# Autodesk Inventor assembly: FinalAssembly
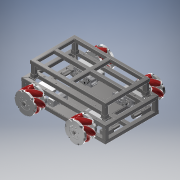
[picture p0: Inventor's stored thumbnail of the model, 180x180]
Saved by Autodesk Inventor 2018 (Build 220112000, 112)
## iProperties
Created: 2018-05-29
Part Number: FinalAssembly
Document SubType Name: Assembly
Designer: P136265
Author: P136265
## Documents named in this file (23)
- C:\Users\P136265\Documents\GitHub\mecanum-cad\FinalAssembly.iam
- C:\Users\P136265\Documents\GitHub\mecanum-cad\MecanumFrame2.iam
- C:\Users\P136265\Documents\GitHub\mecanum-cad\BearingHousing.iam
- C:\Users\P136265\Documents\GitHub\mecanum-cad\WheelShaft.ipt
- C:\Users\P136265\Documents\Inventor\Content Center Files\R2018\en-US\AS 1110\AS 1110 - M8 x 50.ipt
- C:\Users\P136265\Documents\Inventor\Content Center Files\R2018\en-US\AS 1112 (2)\AS 1112 - M8  Type 8.ipt
- C:\Users\P136265\Documents\GitHub\mecanum-cad\WheelKey.ipt
- C:\Users\P136265\Documents\GitHub\mecanum-cad\PulleyKey.ipt
- C:\Users\P136265\Documents\GitHub\mecanum-cad\Mecanum_Assembly.iam
- C:\Users\P136265\Documents\GitHub\mecanum-cad\LiftBase.ipt
- C:\Users\P136265\Documents\GitHub\mecanum-cad\mount.ipt
- C:\Users\P136265\Documents\GitHub\mecanum-cad\Nema 23 Stepper Motor Bipolar L=56mm w Gear Ratio 41 Planetary Gearbox.ipt
- C:\Users\P136265\Documents\GitHub\mecanum-cad\Synchronous Belt1.ipt
- C:\Users\P136265\Documents\GitHub\mecanum-cad\Synchronous Pulley21.ipt
- C:\Users\P136265\Documents\GitHub\mecanum-cad\Synchronous Pulley11.ipt
- C:\Users\P136265\Documents\Inventor\Content Center Files\R2018\en-US\BS EN 24035\ISO 4035 - M20BS EN.ipt
- C:\Users\P136265\Documents\Inventor\Content Center Files\R2018\en-US\BS EN 24035\ISO 4035 - M12BS EN.ipt
- C:\Users\P136265\Documents\GitHub\mecanum-cad\TS-58GZ868D_Open.ipt
- C:\Users\P136265\Documents\GitHub\mecanum-cad\12mm Ball Screw.ipt
- C:\Users\P136265\Documents\GitHub\mecanum-cad\16mm Lead Nut.ipt
- C:\Users\P136265\Documents\GitHub\mecanum-cad\LiftPlate.iam
- C:\Users\P136265\Documents\GitHub\mecanum-cad\LiftPlate_Mount.ipt
- C:\Users\P136265\Documents\Inventor\Content Center Files\R2018\en-US\AS 1110\AS 1110 - M3 x 6.ipt
## Components (119 placed, 22 different names)
1. MecanumFrame2:1 [sub-assembly] — Mate:1, Mate:2, Mate:3, Mate:4, Mate:5, Mate:6, Mate:7, Mate:8, Mate:9, Mate:10, Mate:11, Mate:12, Mate:13, Mate:14, Mate:15, Mate:24, Mate:25, Mate:26, Mate:27, Mate:28, Mate:29, Mate:30, Mate:31, Mate:32, Mate:33, Mate:34, Mate:35, Mate:36, Mate:37, Insert:1, Mate:38, Mate:39, Mate:40, Mate:41, Insert:2, Insert:3, Insert:4, Insert:5, Insert:6, Insert:7, Mate:106, Mate:107, Mate:108, Angle:5, Angle:8, Mate:185, Mate:186, Mate:187, Mate:188, Angle:15, Mate:191, Mate:192
2. BearingHousing:1 [sub-assembly] — Mate:4, Mate:5, Mate:6, Mate:16, Mate:17, Mate:43, Mate:45, Mate:47, Mate:49, Mate:156
3. BearingHousing:2 [sub-assembly] — Mate:7, Mate:8, Mate:9, Mate:18, Mate:19, Mate:51, Mate:53, Mate:55, Mate:57, Mate:154
4. BearingHousing:3 [sub-assembly] — Mate:10, Mate:11, Mate:12, Mate:20, Mate:21, Mate:67, Mate:69, Mate:71, Mate:73, Mate:150
5. BearingHousing:4 [sub-assembly] — Mate:13, Mate:14, Mate:15, Mate:22, Mate:23, Mate:59, Mate:61, Mate:63, Mate:65, Mate:152
6. WheelShaft:1 — Mate:16, Mate:17, Mate:77, Mate:78, Mate:79, Mate:89, Mate:90, Mate:91, Mate:98, Mate:99, Mate:134, Mate:137, Flush:8, Mate:141, Mate:155, Mate:157
7. WheelShaft:2 — Mate:18, Mate:19, Mate:74, Mate:75, Mate:76, Mate:92, Mate:93, Mate:94, Mate:100, Mate:101, Mate:131, Mate:136, Flush:7, Mate:143, Mate:153, Mate:163
8. WheelShaft:3 — Mate:20, Mate:21, Mate:83, Mate:84, Mate:85, Mate:86, Mate:87, Mate:88, Mate:104, Mate:105, Mate:116, Mate:118, Flush:1, Mate:147, Mate:149, Mate:159
9. WheelShaft:4 — Mate:22, Mate:23, Mate:80, Mate:81, Mate:82, Mate:95, Mate:96, Mate:97, Mate:102, Mate:103, Mate:129, Mate:135, Flush:6, Mate:145, Mate:151, Mate:161
10. AS 1110 - Metric M8 x 50:1 — Mate:24, Mate:25, Mate:42
11. AS 1110 - Metric M8 x 50:2 — Mate:26, Mate:27, Mate:44
12. AS 1110 - Metric M8 x 50:3 — Mate:28, Mate:29, Mate:50
13. AS 1110 - Metric M8 x 50:4 — Mate:30, Mate:31, Mate:54
14. AS 1110 - Metric M8 x 50:5 — Mate:32, Mate:33, Mate:56
15. AS 1110 - Metric M8 x 50:6 — Mate:34, Mate:35, Mate:52
16. AS 1110 - Metric M8 x 50:7 — Mate:36, Mate:37, Mate:46
17. AS 1110 - Metric M8 x 50:8 — Insert:1, Mate:48
18. AS 1110 - Metric M8 x 50:9 — Mate:38, Mate:39, Mate:72
19. AS 1110 - Metric M8 x 50:10 — Mate:40, Mate:41, Mate:68
20. AS 1110 - Metric M8 x 50:11 — Insert:2, Mate:64
21. AS 1110 - Metric M8 x 50:12 — Insert:3, Mate:60
22. AS 1110 - Metric M8 x 50:13 — Insert:4, Mate:58
23. AS 1110 - Metric M8 x 50:14 — Insert:5, Mate:62
24. AS 1110 - Metric M8 x 50:15 — Insert:6, Mate:66
25. AS 1110 - Metric M8 x 50:16 — Insert:7, Mate:70
26. AS 1112 (2) - Metric M8  Type 8:1 — Mate:42, Mate:43
27. AS 1112 (2) - Metric M8  Type 8:2 — Mate:44, Mate:45
28. AS 1112 (2) - Metric M8  Type 8:3 — Mate:46, Mate:47
29. AS 1112 (2) - Metric M8  Type 8:4 — Mate:48, Mate:49
30. AS 1112 (2) - Metric M8  Type 8:5 — Mate:50, Mate:51
31. AS 1112 (2) - Metric M8  Type 8:6 — Mate:52, Mate:53
32. AS 1112 (2) - Metric M8  Type 8:7 — Mate:54, Mate:55
33. AS 1112 (2) - Metric M8  Type 8:8 — Mate:56, Mate:57
34. AS 1112 (2) - Metric M8  Type 8:9 — Mate:58, Mate:59
35. AS 1112 (2) - Metric M8  Type 8:10 — Mate:60, Mate:61
36. AS 1112 (2) - Metric M8  Type 8:11 — Mate:62, Mate:63
37. AS 1112 (2) - Metric M8  Type 8:12 — Mate:64, Mate:65
38. AS 1112 (2) - Metric M8  Type 8:13 — Mate:66, Mate:67
39. AS 1112 (2) - Metric M8  Type 8:14 — Mate:68, Mate:69
40. AS 1112 (2) - Metric M8  Type 8:15 — Mate:70, Mate:71
41. AS 1112 (2) - Metric M8  Type 8:16 — Mate:72, Mate:73
42. WheelKey:1 — Mate:74, Mate:75, Mate:76, Angle:2
43. WheelKey:2 — Mate:77, Mate:78, Mate:79, Angle:1
44. WheelKey:3 — Mate:80, Mate:81, Mate:82, Angle:3
45. WheelKey:4 — Mate:83, Mate:84, Mate:85, Angle:4
46. PulleyKey:1 — Mate:86, Mate:87, Mate:88, Angle:6
47. PulleyKey:2 — Mate:89, Mate:90, Mate:91, Angle:9
48. PulleyKey:3 — Mate:92, Mate:93, Mate:94, Angle:10
49. PulleyKey:4 — Mate:95, Mate:96, Mate:97, Angle:11
50. Mecanum_Assembly:1 [sub-assembly] — Mate:98, Angle:1, Mate:99, Mate:142
51. Mecanum_Assembly:2 [sub-assembly] — Mate:100, Angle:2, Mate:101, Mate:144
52. Mecanum_Assembly:3 [sub-assembly] — Mate:104, Angle:4, Mate:105, Mate:148
53. Mecanum_Assembly:4 [sub-assembly] — Mate:102, Angle:3, Mate:103, Mate:146
54. LiftBase:1 — Mate:106, Mate:107, Mate:108, Mate:109, Mate:110, Mate:111, Mate:112, Mate:214, Mate:216, Mate:218, Mate:220, Mate:222, Mate:224, Mate:226, Mate:228, Mate:230, Mate:232, Mate:234, Mate:236, Mate:238, Mate:240, Mate:242, Mate:244
55. mount:1 — Mate:109, Mate:126, Mate:127, Mate:128, Mate:223, Mate:225, Mate:227, Mate:229
56. mount:2 — Mate:110, Mate:120, Mate:121, Mate:122, Mate:239, Mate:241, Mate:243, Mate:245
57. mount:3 — Mate:111, Mate:123, Mate:124, Mate:125, Mate:215, Mate:217, Mate:219, Mate:221
58. mount:4 — Mate:112, Mate:113, Mate:114, Mate:115, Mate:231, Mate:233, Mate:235, Mate:237
59. Nema 23 Stepper Motor Bipolar L=56mm w Gear Ratio 41 Planetary Gearbox:1 — Mate:113, Mate:114, Mate:115, Angle:5, Mate:117, Mate:119, Flush:3, Flush:4
60. Nema 23 Stepper Motor Bipolar L=56mm w Gear Ratio 41 Planetary Gearbox:2 — Mate:123, Mate:124, Mate:125, Flush:5, Mate:133, Mate:140, Flush:16
61. Nema 23 Stepper Motor Bipolar L=56mm w Gear Ratio 41 Planetary Gearbox:3 — Mate:126, Mate:127, Mate:128, Angle:8, Mate:132, Flush:5, Mate:139
62. Nema 23 Stepper Motor Bipolar L=56mm w Gear Ratio 41 Planetary Gearbox:4 — Mate:120, Mate:121, Mate:122, Flush:4, Mate:130, Mate:138
63. Synchronous Belt:1 — Mate:116, Mate:117, Flush:14
64. Synchronous Belt:2 — Mate:131, Mate:132, Flush:12
65. Synchronous Belt:3 — Mate:133, Mate:134, Flush:15
66. Synchronous Belt:4 — Mate:129, Mate:130, Flush:13
67. Synchronous Pulley2:1 — Mate:118, Angle:6, Flush:1, Angle:7, Flush:2, Flush:14, Mate:160
68. Synchronous Pulley2:2 — Mate:135, Flush:6, Angle:11, Flush:9, Angle:13, Mate:162
69. Synchronous Pulley2:3 — Mate:136, Flush:7, Angle:10, Flush:10, Angle:14, Mate:164
70. Synchronous Pulley2:4 — Mate:137, Flush:8, Angle:9, Flush:11, Angle:12, Flush:15, Mate:158
71. Synchronous Pulley1:1 — Mate:119, Angle:7, Flush:2, Flush:3
72. Synchronous Pulley1:2 — Mate:139, Flush:10, Angle:14, Flush:12
73. Synchronous Pulley1:3 — Mate:140, Flush:11, Angle:12, Flush:16
74. Synchronous Pulley1:4 — Mate:138, Flush:9, Angle:13, Flush:13
75. BS EN 24035 - Metric M20:1 — Mate:141, Mate:142
76. BS EN 24035 - Metric M20:2 — Mate:143, Mate:144
77. BS EN 24035 - Metric M20:3 — Mate:145, Mate:146
78. BS EN 24035 - Metric M20:4 — Mate:147, Mate:148
79. BS EN 24035 - Metric M20:5 — Mate:149, Mate:150
80. BS EN 24035 - Metric M20:6 — Mate:151, Mate:152
81. BS EN 24035 - Metric M20:7 — Mate:153, Mate:154
82. BS EN 24035 - Metric M20:8 — Mate:155, Mate:156
83. BS EN 24035 - Metric M12:1 — Mate:157, Mate:158
84. BS EN 24035 - Metric M12:2 — Mate:159, Mate:160
85. BS EN 24035 - Metric M12:3 — Mate:161, Mate:162
86. BS EN 24035 - Metric M12:4 — Mate:163, Mate:164
87. TS-58GZ868D_Open:1 — Mate:165, Flush:19
88. TS-58GZ868D_Open:2 — Mate:166, Mate:169
89. TS-58GZ868D_Open:3 — Mate:167, Flush:18
90. TS-58GZ868D_Open:4 — Mate:168, Flush:17
91. 12mm Ball Screw:1 — Mate:165, Flush:19, Mate:170, Flush:20, Mate:185
92. 12mm Ball Screw:2 — Mate:166, Mate:169, Mate:171, Flush:23, Mate:186
93. 12mm Ball Screw:3 — Mate:167, Flush:18, Mate:172, Flush:21, Mate:187
94. 12mm Ball Screw:4 — Mate:168, Flush:17, Mate:173, Flush:22, Mate:188
95. 16mm Lead Nut:1 — Mate:170, Flush:20, Flush:26, Flush:27, Mate:207, Mate:208
96. 16mm Lead Nut:2 — Mate:171, Flush:23, Flush:25, Flush:27, Mate:196, Mate:197
97. 16mm Lead Nut:3 — Mate:172, Flush:21, Flush:24, Flush:26, Mate:209, Mate:210
98. 16mm Lead Nut:4 — Mate:173, Flush:22, Flush:24, Flush:25, Mate:211, Mate:212, Mate:213
99. LiftPlate:1 [sub-assembly] — Angle:15, Mate:191, Mate:192, Mate:193, Mate:194, Mate:195, Mate:198, Mate:199, Mate:200, Mate:201, Mate:202, Mate:203, Mate:204, Mate:205, Mate:206
100. LiftPlate_Mount:1 — Mate:193, Mate:194, Mate:195, Mate:196, Mate:197
101. LiftPlate_Mount:2 — Mate:201, Mate:202, Mate:203, Mate:209, Mate:210
102. LiftPlate_Mount:3 — Mate:204, Mate:205, Mate:206, Mate:207, Mate:208
103. LiftPlate_Mount:4 — Mate:198, Mate:199, Mate:200, Mate:211, Mate:212, Mate:213
104. AS 1110 - Metric M3 x 6:1 — Mate:214, Mate:215
105. AS 1110 - Metric M3 x 6:2 — Mate:216, Mate:217
106. AS 1110 - Metric M3 x 6:3 — Mate:218, Mate:219
107. AS 1110 - Metric M3 x 6:4 — Mate:220, Mate:221
108. AS 1110 - Metric M3 x 6:5 — Mate:222, Mate:223
109. AS 1110 - Metric M3 x 6:6 — Mate:224, Mate:225
110. AS 1110 - Metric M3 x 6:7 — Mate:226, Mate:227
111. AS 1110 - Metric M3 x 6:8 — Mate:228, Mate:229
112. AS 1110 - Metric M3 x 6:9 — Mate:230, Mate:231
113. AS 1110 - Metric M3 x 6:10 — Mate:232, Mate:233
114. AS 1110 - Metric M3 x 6:11 — Mate:234, Mate:235
115. AS 1110 - Metric M3 x 6:12 — Mate:236, Mate:237
116. AS 1110 - Metric M3 x 6:13 — Mate:238, Mate:239
117. AS 1110 - Metric M3 x 6:14 — Mate:240, Mate:241
118. AS 1110 - Metric M3 x 6:15 — Mate:242, Mate:243
119. AS 1110 - Metric M3 x 6:16 — Mate:244, Mate:245
## Relationships (281: Mate 232, Flush 27, Angle 15, Insert 7)
- Mate:1: MecanumFrame2:1
- Mate:2: MecanumFrame2:1
- Mate:3: MecanumFrame2:1
- Mate:4: MecanumFrame2:1 ↔ BearingHousing:1
- Mate:5: MecanumFrame2:1 ↔ BearingHousing:1
- Mate:6: MecanumFrame2:1 ↔ BearingHousing:1
- Mate:7: MecanumFrame2:1 ↔ BearingHousing:2
- Mate:8: MecanumFrame2:1 ↔ BearingHousing:2
- Mate:9: MecanumFrame2:1 ↔ BearingHousing:2
- Mate:10: MecanumFrame2:1 ↔ BearingHousing:3
- Mate:11: MecanumFrame2:1 ↔ BearingHousing:3
- Mate:12: MecanumFrame2:1 ↔ BearingHousing:3
- Mate:13: MecanumFrame2:1 ↔ BearingHousing:4
- Mate:14: MecanumFrame2:1 ↔ BearingHousing:4
- Mate:15: MecanumFrame2:1 ↔ BearingHousing:4
- Mate:16: BearingHousing:1 ↔ WheelShaft:1
- Mate:17: BearingHousing:1 ↔ WheelShaft:1
- Mate:18: BearingHousing:2 ↔ WheelShaft:2
- Mate:19: BearingHousing:2 ↔ WheelShaft:2
- Mate:20: BearingHousing:3 ↔ WheelShaft:3
- Mate:21: BearingHousing:3 ↔ WheelShaft:3
- Mate:22: BearingHousing:4 ↔ WheelShaft:4
- Mate:23: BearingHousing:4 ↔ WheelShaft:4
- Mate:24: MecanumFrame2:1 ↔ AS 1110 - Metric M8 x 50:1
- Mate:25: MecanumFrame2:1 ↔ AS 1110 - Metric M8 x 50:1
- Mate:26: MecanumFrame2:1 ↔ AS 1110 - Metric M8 x 50:2
- Mate:27: MecanumFrame2:1 ↔ AS 1110 - Metric M8 x 50:2
- Mate:28: MecanumFrame2:1 ↔ AS 1110 - Metric M8 x 50:3
- Mate:29: MecanumFrame2:1 ↔ AS 1110 - Metric M8 x 50:3
- Mate:30: MecanumFrame2:1 ↔ AS 1110 - Metric M8 x 50:4
- Mate:31: MecanumFrame2:1 ↔ AS 1110 - Metric M8 x 50:4
- Mate:32: MecanumFrame2:1 ↔ AS 1110 - Metric M8 x 50:5
- Mate:33: MecanumFrame2:1 ↔ AS 1110 - Metric M8 x 50:5
- Mate:34: MecanumFrame2:1 ↔ AS 1110 - Metric M8 x 50:6
- Mate:35: MecanumFrame2:1 ↔ AS 1110 - Metric M8 x 50:6
- Mate:36: MecanumFrame2:1 ↔ AS 1110 - Metric M8 x 50:7
- Mate:37: MecanumFrame2:1 ↔ AS 1110 - Metric M8 x 50:7
- Insert:1: MecanumFrame2:1 ↔ AS 1110 - Metric M8 x 50:8
- Mate:38: MecanumFrame2:1 ↔ AS 1110 - Metric M8 x 50:9
- Mate:39: MecanumFrame2:1 ↔ AS 1110 - Metric M8 x 50:9
- Mate:40: MecanumFrame2:1 ↔ AS 1110 - Metric M8 x 50:10
- Mate:41: MecanumFrame2:1 ↔ AS 1110 - Metric M8 x 50:10
- Insert:2: MecanumFrame2:1 ↔ AS 1110 - Metric M8 x 50:11
- Insert:3: MecanumFrame2:1 ↔ AS 1110 - Metric M8 x 50:12
- Insert:4: MecanumFrame2:1 ↔ AS 1110 - Metric M8 x 50:13
- Insert:5: MecanumFrame2:1 ↔ AS 1110 - Metric M8 x 50:14
- Insert:6: MecanumFrame2:1 ↔ AS 1110 - Metric M8 x 50:15
- Insert:7: MecanumFrame2:1 ↔ AS 1110 - Metric M8 x 50:16
- Mate:42: AS 1110 - Metric M8 x 50:1 ↔ AS 1112 (2) - Metric M8  Type 8:1
- Mate:43: BearingHousing:1 ↔ AS 1112 (2) - Metric M8  Type 8:1
- Mate:44: AS 1110 - Metric M8 x 50:2 ↔ AS 1112 (2) - Metric M8  Type 8:2
- Mate:45: BearingHousing:1 ↔ AS 1112 (2) - Metric M8  Type 8:2
- Mate:46: AS 1110 - Metric M8 x 50:7 ↔ AS 1112 (2) - Metric M8  Type 8:3
- Mate:47: BearingHousing:1 ↔ AS 1112 (2) - Metric M8  Type 8:3
- Mate:48: AS 1110 - Metric M8 x 50:8 ↔ AS 1112 (2) - Metric M8  Type 8:4
- Mate:49: BearingHousing:1 ↔ AS 1112 (2) - Metric M8  Type 8:4
- Mate:50: AS 1110 - Metric M8 x 50:3 ↔ AS 1112 (2) - Metric M8  Type 8:5
- Mate:51: BearingHousing:2 ↔ AS 1112 (2) - Metric M8  Type 8:5
- Mate:52: AS 1110 - Metric M8 x 50:6 ↔ AS 1112 (2) - Metric M8  Type 8:6
- Mate:53: BearingHousing:2 ↔ AS 1112 (2) - Metric M8  Type 8:6
- Mate:54: AS 1110 - Metric M8 x 50:4 ↔ AS 1112 (2) - Metric M8  Type 8:7
- Mate:55: BearingHousing:2 ↔ AS 1112 (2) - Metric M8  Type 8:7
- Mate:56: AS 1110 - Metric M8 x 50:5 ↔ AS 1112 (2) - Metric M8  Type 8:8
- Mate:57: BearingHousing:2 ↔ AS 1112 (2) - Metric M8  Type 8:8
- Mate:58: AS 1110 - Metric M8 x 50:13 ↔ AS 1112 (2) - Metric M8  Type 8:9
- Mate:59: BearingHousing:4 ↔ AS 1112 (2) - Metric M8  Type 8:9
- Mate:60: AS 1110 - Metric M8 x 50:12 ↔ AS 1112 (2) - Metric M8  Type 8:10
- Mate:61: BearingHousing:4 ↔ AS 1112 (2) - Metric M8  Type 8:10
- Mate:62: AS 1110 - Metric M8 x 50:14 ↔ AS 1112 (2) - Metric M8  Type 8:11
- Mate:63: BearingHousing:4 ↔ AS 1112 (2) - Metric M8  Type 8:11
- Mate:64: AS 1110 - Metric M8 x 50:11 ↔ AS 1112 (2) - Metric M8  Type 8:12
- Mate:65: BearingHousing:4 ↔ AS 1112 (2) - Metric M8  Type 8:12
- Mate:66: AS 1110 - Metric M8 x 50:15 ↔ AS 1112 (2) - Metric M8  Type 8:13
- Mate:67: BearingHousing:3 ↔ AS 1112 (2) - Metric M8  Type 8:13
- Mate:68: AS 1110 - Metric M8 x 50:10 ↔ AS 1112 (2) - Metric M8  Type 8:14
- Mate:69: BearingHousing:3 ↔ AS 1112 (2) - Metric M8  Type 8:14
- Mate:70: AS 1110 - Metric M8 x 50:16 ↔ AS 1112 (2) - Metric M8  Type 8:15
- Mate:71: BearingHousing:3 ↔ AS 1112 (2) - Metric M8  Type 8:15
- Mate:72: AS 1110 - Metric M8 x 50:9 ↔ AS 1112 (2) - Metric M8  Type 8:16
- Mate:73: BearingHousing:3 ↔ AS 1112 (2) - Metric M8  Type 8:16
- Mate:74: WheelShaft:2 ↔ WheelKey:1
- Mate:75: WheelShaft:2 ↔ WheelKey:1
- Mate:76: WheelShaft:2 ↔ WheelKey:1
- Mate:77: WheelShaft:1 ↔ WheelKey:2
- Mate:78: WheelShaft:1 ↔ WheelKey:2
- Mate:79: WheelShaft:1 ↔ WheelKey:2
- Mate:80: WheelShaft:4 ↔ WheelKey:3
- Mate:81: WheelShaft:4 ↔ WheelKey:3
- Mate:82: WheelShaft:4 ↔ WheelKey:3
- Mate:83: WheelShaft:3 ↔ WheelKey:4
- Mate:84: WheelShaft:3 ↔ WheelKey:4
- Mate:85: WheelShaft:3 ↔ WheelKey:4
- Mate:86: WheelShaft:3 ↔ PulleyKey:1
- Mate:87: WheelShaft:3 ↔ PulleyKey:1
- Mate:88: WheelShaft:3 ↔ PulleyKey:1
- Mate:89: WheelShaft:1 ↔ PulleyKey:2
- Mate:90: WheelShaft:1 ↔ PulleyKey:2
- Mate:91: WheelShaft:1 ↔ PulleyKey:2
- Mate:92: WheelShaft:2 ↔ PulleyKey:3
- Mate:93: WheelShaft:2 ↔ PulleyKey:3
- Mate:94: WheelShaft:2 ↔ PulleyKey:3
- Mate:95: WheelShaft:4 ↔ PulleyKey:4
- Mate:96: WheelShaft:4 ↔ PulleyKey:4
- Mate:97: WheelShaft:4 ↔ PulleyKey:4
- Mate:98: WheelShaft:1 ↔ Mecanum_Assembly:1
- Angle:1 (0 deg): WheelKey:2 ↔ Mecanum_Assembly:1
- Mate:99: WheelShaft:1 ↔ Mecanum_Assembly:1
- Mate:100: WheelShaft:2 ↔ Mecanum_Assembly:2
- Angle:2 (0 deg): WheelKey:1 ↔ Mecanum_Assembly:2
- Mate:101: WheelShaft:2 ↔ Mecanum_Assembly:2
- Mate:102: WheelShaft:4 ↔ Mecanum_Assembly:4
- Angle:3 (0 deg): WheelKey:3 ↔ Mecanum_Assembly:4
- Mate:103: WheelShaft:4 ↔ Mecanum_Assembly:4
- Mate:104: WheelShaft:3 ↔ Mecanum_Assembly:3
- Angle:4 (0 deg): WheelKey:4 ↔ Mecanum_Assembly:3
- Mate:105: WheelShaft:3 ↔ Mecanum_Assembly:3
- Mate:106: MecanumFrame2:1 ↔ LiftBase:1
- Mate:107: MecanumFrame2:1 ↔ LiftBase:1
- Mate:108: MecanumFrame2:1 ↔ LiftBase:1
- Mate:109: LiftBase:1 ↔ mount:1
- Mate:110: LiftBase:1 ↔ mount:2
- Mate:111: LiftBase:1 ↔ mount:3
- Mate:112: LiftBase:1 ↔ mount:4
- Mate:113: mount:4 ↔ Nema 23 Stepper Motor Bipolar L=56mm w Gear Ratio 41 Planetary Gearbox:1
- Mate:114: mount:4 ↔ Nema 23 Stepper Motor Bipolar L=56mm w Gear Ratio 41 Planetary Gearbox:1
- Mate:115: mount:4 ↔ Nema 23 Stepper Motor Bipolar L=56mm w Gear Ratio 41 Planetary Gearbox:1
- Angle:5 (0 deg): MecanumFrame2:1 ↔ Nema 23 Stepper Motor Bipolar L=56mm w Gear Ratio 41 Planetary Gearbox:1
- Mate:116: WheelShaft:3 ↔ Synchronous Belt:1
- Mate:117: Nema 23 Stepper Motor Bipolar L=56mm w Gear Ratio 41 Planetary Gearbox:1 ↔ Synchronous Belt:1
- Mate:118: WheelShaft:3 ↔ Synchronous Pulley2:1
- Angle:6 (0 deg): PulleyKey:1 ↔ Synchronous Pulley2:1
- Flush:1 (10 mm): WheelShaft:3 ↔ Synchronous Pulley2:1
- Mate:119: Nema 23 Stepper Motor Bipolar L=56mm w Gear Ratio 41 Planetary Gearbox:1 ↔ Synchronous Pulley1:1
- Angle:7 (0 deg): Synchronous Pulley2:1 ↔ Synchronous Pulley1:1
- Flush:2: Synchronous Pulley2:1 ↔ Synchronous Pulley1:1
- Flush:3: Nema 23 Stepper Motor Bipolar L=56mm w Gear Ratio 41 Planetary Gearbox:1 ↔ Synchronous Pulley1:1
- Mate:120: mount:2 ↔ Nema 23 Stepper Motor Bipolar L=56mm w Gear Ratio 41 Planetary Gearbox:4
- Mate:121: mount:2 ↔ Nema 23 Stepper Motor Bipolar L=56mm w Gear Ratio 41 Planetary Gearbox:4
- Mate:122: mount:2 ↔ Nema 23 Stepper Motor Bipolar L=56mm w Gear Ratio 41 Planetary Gearbox:4
- Mate:123: mount:3 ↔ Nema 23 Stepper Motor Bipolar L=56mm w Gear Ratio 41 Planetary Gearbox:2
- Mate:124: mount:3 ↔ Nema 23 Stepper Motor Bipolar L=56mm w Gear Ratio 41 Planetary Gearbox:2
- Mate:125: mount:3 ↔ Nema 23 Stepper Motor Bipolar L=56mm w Gear Ratio 41 Planetary Gearbox:2
- Mate:126: mount:1 ↔ Nema 23 Stepper Motor Bipolar L=56mm w Gear Ratio 41 Planetary Gearbox:3
- Mate:127: mount:1 ↔ Nema 23 Stepper Motor Bipolar L=56mm w Gear Ratio 41 Planetary Gearbox:3
- Mate:128: mount:1 ↔ Nema 23 Stepper Motor Bipolar L=56mm w Gear Ratio 41 Planetary Gearbox:3
- Flush:4: Nema 23 Stepper Motor Bipolar L=56mm w Gear Ratio 41 Planetary Gearbox:1 ↔ Nema 23 Stepper Motor Bipolar L=56mm w Gear Ratio 41 Planetary Gearbox:4
- Mate:129: WheelShaft:4 ↔ Synchronous Belt:4
- Mate:130: Nema 23 Stepper Motor Bipolar L=56mm w Gear Ratio 41 Planetary Gearbox:4 ↔ Synchronous Belt:4
- Angle:8 (0 deg): MecanumFrame2:1 ↔ Nema 23 Stepper Motor Bipolar L=56mm w Gear Ratio 41 Planetary Gearbox:3
- Mate:131: WheelShaft:2 ↔ Synchronous Belt:2
- Mate:132: Nema 23 Stepper Motor Bipolar L=56mm w Gear Ratio 41 Planetary Gearbox:3 ↔ Synchronous Belt:2
- Flush:5: Nema 23 Stepper Motor Bipolar L=56mm w Gear Ratio 41 Planetary Gearbox:2 ↔ Nema 23 Stepper Motor Bipolar L=56mm w Gear Ratio 41 Planetary Gearbox:3
- Mate:133: Nema 23 Stepper Motor Bipolar L=56mm w Gear Ratio 41 Planetary Gearbox:2 ↔ Synchronous Belt:3
- Mate:134: WheelShaft:1 ↔ Synchronous Belt:3
- Mate:135: WheelShaft:4 ↔ Synchronous Pulley2:2
- Flush:6 (10 mm): WheelShaft:4 ↔ Synchronous Pulley2:2
- Mate:136: WheelShaft:2 ↔ Synchronous Pulley2:3
- Flush:7 (10 mm): WheelShaft:2 ↔ Synchronous Pulley2:3
- Mate:137: WheelShaft:1 ↔ Synchronous Pulley2:4
- Flush:8 (10 mm): WheelShaft:1 ↔ Synchronous Pulley2:4
- Angle:9 (0 deg): PulleyKey:2 ↔ Synchronous Pulley2:4
- Angle:10 (0 deg): PulleyKey:3 ↔ Synchronous Pulley2:3
- Angle:11 (0 deg): PulleyKey:4 ↔ Synchronous Pulley2:2
- Mate:138: Nema 23 Stepper Motor Bipolar L=56mm w Gear Ratio 41 Planetary Gearbox:4 ↔ Synchronous Pulley1:4
- Flush:9: Synchronous Pulley2:2 ↔ Synchronous Pulley1:4
- Mate:139: Nema 23 Stepper Motor Bipolar L=56mm w Gear Ratio 41 Planetary Gearbox:3 ↔ Synchronous Pulley1:2
- Flush:10: Synchronous Pulley2:3 ↔ Synchronous Pulley1:2
- Mate:140: Nema 23 Stepper Motor Bipolar L=56mm w Gear Ratio 41 Planetary Gearbox:2 ↔ Synchronous Pulley1:3
- Flush:11: Synchronous Pulley2:4 ↔ Synchronous Pulley1:3
- Angle:12 (0 deg): Synchronous Pulley2:4 ↔ Synchronous Pulley1:3
- Angle:13 (0 deg): Synchronous Pulley2:2 ↔ Synchronous Pulley1:4
- Angle:14 (0 deg): Synchronous Pulley2:3 ↔ Synchronous Pulley1:2
- Flush:12 (1.5 mm): Synchronous Belt:2 ↔ Synchronous Pulley1:2
- Flush:13 (1.5 mm): Synchronous Belt:4 ↔ Synchronous Pulley1:4
- Flush:14 (1.5 mm): Synchronous Belt:1 ↔ Synchronous Pulley2:1
- Flush:15 (1.5 mm): Synchronous Belt:3 ↔ Synchronous Pulley2:4
- Flush:16: Nema 23 Stepper Motor Bipolar L=56mm w Gear Ratio 41 Planetary Gearbox:2 ↔ Synchronous Pulley1:3
- Mate:141: WheelShaft:1 ↔ BS EN 24035 - Metric M20:1
- Mate:142: Mecanum_Assembly:1 ↔ BS EN 24035 - Metric M20:1
- Mate:143: WheelShaft:2 ↔ BS EN 24035 - Metric M20:2
- Mate:144: Mecanum_Assembly:2 ↔ BS EN 24035 - Metric M20:2
- Mate:145: WheelShaft:4 ↔ BS EN 24035 - Metric M20:3
- Mate:146: Mecanum_Assembly:4 ↔ BS EN 24035 - Metric M20:3
- Mate:147: WheelShaft:3 ↔ BS EN 24035 - Metric M20:4
- Mate:148: Mecanum_Assembly:3 ↔ BS EN 24035 - Metric M20:4
- Mate:149: WheelShaft:3 ↔ BS EN 24035 - Metric M20:5
- Mate:150: BearingHousing:3 ↔ BS EN 24035 - Metric M20:5
- Mate:151: WheelShaft:4 ↔ BS EN 24035 - Metric M20:6
- Mate:152: BearingHousing:4 ↔ BS EN 24035 - Metric M20:6
- Mate:153: WheelShaft:2 ↔ BS EN 24035 - Metric M20:7
- Mate:154: BearingHousing:2 ↔ BS EN 24035 - Metric M20:7
- Mate:155: WheelShaft:1 ↔ BS EN 24035 - Metric M20:8
- Mate:156: BearingHousing:1 ↔ BS EN 24035 - Metric M20:8
- Mate:157: WheelShaft:1 ↔ BS EN 24035 - Metric M12:1
- Mate:158: Synchronous Pulley2:4 ↔ BS EN 24035 - Metric M12:1
- Mate:159: WheelShaft:3 ↔ BS EN 24035 - Metric M12:2
- Mate:160: Synchronous Pulley2:1 ↔ BS EN 24035 - Metric M12:2
- Mate:161: WheelShaft:4 ↔ BS EN 24035 - Metric M12:3
- Mate:162: Synchronous Pulley2:2 ↔ BS EN 24035 - Metric M12:3
- Mate:163: WheelShaft:2 ↔ BS EN 24035 - Metric M12:4
- Mate:164: Synchronous Pulley2:3 ↔ BS EN 24035 - Metric M12:4
- Mate:165: TS-58GZ868D_Open:1 ↔ 12mm Ball Screw:1
- Mate:166: TS-58GZ868D_Open:2 ↔ 12mm Ball Screw:2
- Mate:167: TS-58GZ868D_Open:3 ↔ 12mm Ball Screw:3
- Mate:168: TS-58GZ868D_Open:4 ↔ 12mm Ball Screw:4
- Flush:17 (130 mm): TS-58GZ868D_Open:4 ↔ 12mm Ball Screw:4
- Flush:18 (130 mm): TS-58GZ868D_Open:3 ↔ 12mm Ball Screw:3
- Mate:169 (130 mm): TS-58GZ868D_Open:2 ↔ 12mm Ball Screw:2
- Flush:19 (130 mm): TS-58GZ868D_Open:1 ↔ 12mm Ball Screw:1
- Mate:170: 12mm Ball Screw:1 ↔ 16mm Lead Nut:1
- Mate:171: 12mm Ball Screw:2 ↔ 16mm Lead Nut:2
- Mate:172: 12mm Ball Screw:3 ↔ 16mm Lead Nut:3
- Mate:173: 12mm Ball Screw:4 ↔ 16mm Lead Nut:4
- Flush:20: 12mm Ball Screw:1 ↔ 16mm Lead Nut:1
- Flush:21: 12mm Ball Screw:3 ↔ 16mm Lead Nut:3
- Flush:22: 12mm Ball Screw:4 ↔ 16mm Lead Nut:4
- Flush:23: 12mm Ball Screw:2 ↔ 16mm Lead Nut:2
- Flush:24: 16mm Lead Nut:3 ↔ 16mm Lead Nut:4
- Flush:25: 16mm Lead Nut:2 ↔ 16mm Lead Nut:4
- Flush:26: 16mm Lead Nut:1 ↔ 16mm Lead Nut:3
- Flush:27: 16mm Lead Nut:1 ↔ 16mm Lead Nut:2
- Mate:185: MecanumFrame2:1 ↔ 12mm Ball Screw:1
- Mate:186: MecanumFrame2:1 ↔ 12mm Ball Screw:2
- Mate:187: MecanumFrame2:1 ↔ 12mm Ball Screw:3
- Mate:188: MecanumFrame2:1 ↔ 12mm Ball Screw:4
- Angle:15 (0 deg): MecanumFrame2:1 ↔ LiftPlate:1
- Mate:191 (7.5 mm): MecanumFrame2:1 ↔ LiftPlate:1
- Mate:192 (7.5 mm): MecanumFrame2:1 ↔ LiftPlate:1
- Mate:193: LiftPlate:1 ↔ LiftPlate_Mount:1
- Mate:194: LiftPlate:1 ↔ LiftPlate_Mount:1
- Mate:195: LiftPlate:1 ↔ LiftPlate_Mount:1
- Mate:196: 16mm Lead Nut:2 ↔ LiftPlate_Mount:1
- Mate:197: 16mm Lead Nut:2 ↔ LiftPlate_Mount:1
- Mate:198: LiftPlate:1 ↔ LiftPlate_Mount:4
- Mate:199: LiftPlate:1 ↔ LiftPlate_Mount:4
- Mate:200: LiftPlate:1 ↔ LiftPlate_Mount:4
- Mate:201: LiftPlate:1 ↔ LiftPlate_Mount:2
- Mate:202: LiftPlate:1 ↔ LiftPlate_Mount:2
- Mate:203: LiftPlate:1 ↔ LiftPlate_Mount:2
- Mate:204: LiftPlate:1 ↔ LiftPlate_Mount:3
- Mate:205: LiftPlate:1 ↔ LiftPlate_Mount:3
- Mate:206: LiftPlate:1 ↔ LiftPlate_Mount:3
- Mate:207: 16mm Lead Nut:1 ↔ LiftPlate_Mount:3
- Mate:208: 16mm Lead Nut:1 ↔ LiftPlate_Mount:3
- Mate:209: 16mm Lead Nut:3 ↔ LiftPlate_Mount:2
- Mate:210: 16mm Lead Nut:3 ↔ LiftPlate_Mount:2
- Mate:211: 16mm Lead Nut:4 ↔ LiftPlate_Mount:4
- Mate:212: 16mm Lead Nut:4 ↔ LiftPlate_Mount:4
- Mate:213: 16mm Lead Nut:4 ↔ LiftPlate_Mount:4
- Mate:214: LiftBase:1 ↔ AS 1110 - Metric M3 x 6:1
- Mate:215: mount:3 ↔ AS 1110 - Metric M3 x 6:1
- Mate:216: LiftBase:1 ↔ AS 1110 - Metric M3 x 6:2
- Mate:217: mount:3 ↔ AS 1110 - Metric M3 x 6:2
- Mate:218: LiftBase:1 ↔ AS 1110 - Metric M3 x 6:3
- Mate:219: mount:3 ↔ AS 1110 - Metric M3 x 6:3
- Mate:220: LiftBase:1 ↔ AS 1110 - Metric M3 x 6:4
- Mate:221: mount:3 ↔ AS 1110 - Metric M3 x 6:4
- Mate:222: LiftBase:1 ↔ AS 1110 - Metric M3 x 6:5
- Mate:223: mount:1 ↔ AS 1110 - Metric M3 x 6:5
- Mate:224: LiftBase:1 ↔ AS 1110 - Metric M3 x 6:6
- Mate:225: mount:1 ↔ AS 1110 - Metric M3 x 6:6
- Mate:226: LiftBase:1 ↔ AS 1110 - Metric M3 x 6:7
- Mate:227: mount:1 ↔ AS 1110 - Metric M3 x 6:7
- Mate:228: LiftBase:1 ↔ AS 1110 - Metric M3 x 6:8
- Mate:229: mount:1 ↔ AS 1110 - Metric M3 x 6:8
- Mate:230: LiftBase:1 ↔ AS 1110 - Metric M3 x 6:9
- Mate:231: mount:4 ↔ AS 1110 - Metric M3 x 6:9
- Mate:232: LiftBase:1 ↔ AS 1110 - Metric M3 x 6:10
- Mate:233: mount:4 ↔ AS 1110 - Metric M3 x 6:10
- Mate:234: LiftBase:1 ↔ AS 1110 - Metric M3 x 6:11
- Mate:235: mount:4 ↔ AS 1110 - Metric M3 x 6:11
- Mate:236: LiftBase:1 ↔ AS 1110 - Metric M3 x 6:12
- Mate:237: mount:4 ↔ AS 1110 - Metric M3 x 6:12
- Mate:238: LiftBase:1 ↔ AS 1110 - Metric M3 x 6:13
- Mate:239: mount:2 ↔ AS 1110 - Metric M3 x 6:13
- Mate:240: LiftBase:1 ↔ AS 1110 - Metric M3 x 6:14
- Mate:241: mount:2 ↔ AS 1110 - Metric M3 x 6:14
- Mate:242: LiftBase:1 ↔ AS 1110 - Metric M3 x 6:15
- Mate:243: mount:2 ↔ AS 1110 - Metric M3 x 6:15
- Mate:244: LiftBase:1 ↔ AS 1110 - Metric M3 x 6:16
- Mate:245: mount:2 ↔ AS 1110 - Metric M3 x 6:16
